# Autodesk Inventor assembly: Lifting Chasis Assembly Milestone 2
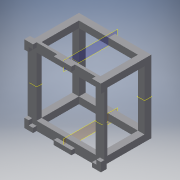
[picture p0: Inventor's stored thumbnail of the model, 180x180]
Saved by Autodesk Inventor 2016 (Build 200138000, 138)
## iProperties
Created: 2016-03-08
Part Number: Lifting Chasis Assembly Milestone 2
Document SubType Name: Assembly
Designer: Kenneth Daniel
Author: Kenneth Daniel
## Documents named in this file (4)
- C:\Users\Kenneth Daniel\Documents\Enes 100A\Lifting Chasis Assembly Milestone 2.iam
- C:\Users\Kenneth Daniel\Documents\Enes 100A\Lifting Chassis Components Milestone 2.ipt
- C:\Users\Kenneth Daniel\Documents\Enes 100A\Lifting Chassis Component Milestone 2.ipt
- C:\Users\Kenneth Daniel\Documents\Enes 100A\Lifting Chasis Component Milestone 2.ipt
## Components (6 placed, 3 different names)
1. Lifting Chassis Components Milestone 2:1 — Mate:1, Mate:2, Mate:3, Mate:4, Mate:5, Mate:6
2. Lifting Chassis Component Milestone 2:1 — Mate:4, Mate:5, Mate:6, Mate:8, Mate:9, Flush:1
3. Lifting Chassis Component Milestone 2:2 — Mate:1, Mate:2, Mate:3, Mate:7
4. Lifting Chassis Components Milestone 2:2 — Mate:7, Mate:8, Mate:9, Flush:1, Mate:10, Mate:11, Mate:12, Mate:13, Mate:14, Mate:15
5. Lifting Chasis Component Milestone 2:1 — Mate:13, Mate:14, Mate:15
6. Lifting Chasis Component Milestone 2:2 — Mate:10, Mate:11, Mate:12
## Relationships (16: Mate 15, Flush 1)
- Mate:1: Lifting Chassis Components Milestone 2:1 ↔ Lifting Chassis Component Milestone 2:2
- Mate:2: Lifting Chassis Components Milestone 2:1 ↔ Lifting Chassis Component Milestone 2:2
- Mate:3: Lifting Chassis Components Milestone 2:1 ↔ Lifting Chassis Component Milestone 2:2
- Mate:4: Lifting Chassis Components Milestone 2:1 ↔ Lifting Chassis Component Milestone 2:1
- Mate:5: Lifting Chassis Components Milestone 2:1 ↔ Lifting Chassis Component Milestone 2:1
- Mate:6: Lifting Chassis Components Milestone 2:1 ↔ Lifting Chassis Component Milestone 2:1
- Mate:7: Lifting Chassis Component Milestone 2:2 ↔ Lifting Chassis Components Milestone 2:2
- Mate:8: Lifting Chassis Component Milestone 2:1 ↔ Lifting Chassis Components Milestone 2:2
- Mate:9: Lifting Chassis Component Milestone 2:1 ↔ Lifting Chassis Components Milestone 2:2
- Flush:1: Lifting Chassis Component Milestone 2:1 ↔ Lifting Chassis Components Milestone 2:2
- Mate:10: Lifting Chassis Components Milestone 2:2 ↔ Lifting Chasis Component Milestone 2:2
- Mate:11: Lifting Chassis Components Milestone 2:2 ↔ Lifting Chasis Component Milestone 2:2
- Mate:12: Lifting Chassis Components Milestone 2:2 ↔ Lifting Chasis Component Milestone 2:2
- Mate:13: Lifting Chassis Components Milestone 2:2 ↔ Lifting Chasis Component Milestone 2:1
- Mate:14: Lifting Chassis Components Milestone 2:2 ↔ Lifting Chasis Component Milestone 2:1
- Mate:15: Lifting Chassis Components Milestone 2:2 ↔ Lifting Chasis Component Milestone 2:1
